# Autodesk Inventor assembly: wheeAndTrackLift
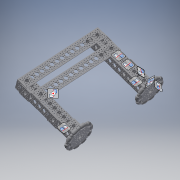
[picture p0: Inventor's stored thumbnail of the model, 180x180]
Saved by Autodesk Inventor 2017 (Build 210142000, 142)
## iProperties
Created: 2017-11-11
Part Number: wheeAndTrackLift
Document SubType Name: Assembly
Designer: User
Author: User
## Documents named in this file (5)
- C:\Robotics\CAD\2017-18_CAD\wheeAndTrackLift.iam
- C:\Robotics\CAD\COTSParts\Actobotics\585 parts\585450.ipt
- C:\Robotics\CAD\COTSParts\Actobotics\585 parts\585424.ipt
- C:\Robotics\CAD\COTSParts\Actobotics\595 parts\595671 Part.ipt
- C:\Robotics\CAD\COTSParts\Actobotics\585 parts\585728.ipt
## Components (12 placed, 4 different names)
1. 585450:1 — Flush:2, Mate:8, Mate:16, Flush:5, Mate:17, Flush:6, Mate:21, Mate:24, Mate:25, Mate:26, Flush:7, Mate:31, Mate:32
2. 585450:2 — Flush:2, Mate:10, Mate:16, Flush:4, Flush:5, Mate:18, Mate:19, Mate:20, Mate:22, Mate:23, Mate:27, Mate:28, Flush:8, Mate:29, Mate:30
3. 585424:1 — Mate:8, Mate:13, Mate:14, Mate:17, Flush:6
4. 585424:2 — Mate:10, Mate:11, Mate:12, Flush:4, Mate:18
5. 595671 Part:1 — Mate:13, Mate:14
6. 595671 Part:2 — Mate:11, Mate:12
7. 585728:1 — Mate:22, Mate:23, Mate:24
8. 585728:2 — Mate:19, Mate:20, Mate:21
9. 585424:3 — Mate:29, Mate:30, Flush:9, Flush:10
10. 585424:4 — Mate:31, Mate:32, Flush:10
11. 585424:5 — Mate:27, Mate:28, Flush:8, Flush:9
12. 585424:6 — Mate:25, Mate:26, Flush:7
## Relationships (31: Mate 23, Flush 8)
- Flush:2: 585450:1 ↔ 585450:2
- Mate:8: 585450:1 ↔ 585424:1
- Mate:10: 585450:2 ↔ 585424:2
- Mate:11: 585424:2 ↔ 595671 Part:2
- Mate:12: 585424:2 ↔ 595671 Part:2
- Mate:13: 585424:1 ↔ 595671 Part:1
- Mate:14: 585424:1 ↔ 595671 Part:1
- Mate:16 (228.6 mm): 585450:1 ↔ 585450:2
- Flush:4: 585450:2 ↔ 585424:2
- Flush:5: 585450:1 ↔ 585450:2
- Mate:17: 585450:1 ↔ 585424:1
- Flush:6: 585450:1 ↔ 585424:1
- Mate:18: 585450:2 ↔ 585424:2
- Mate:19: 585450:2 ↔ 585728:2
- Mate:20: 585450:2 ↔ 585728:2
- Mate:21: 585450:1 ↔ 585728:2
- Mate:22: 585450:2 ↔ 585728:1
- Mate:23: 585450:2 ↔ 585728:1
- Mate:24: 585450:1 ↔ 585728:1
- Mate:25: 585450:1 ↔ 585424:6
- Mate:26: 585450:1 ↔ 585424:6
- Flush:7: 585450:1 ↔ 585424:6
- Mate:27: 585450:2 ↔ 585424:5
- Mate:28: 585450:2 ↔ 585424:5
- Flush:8: 585450:2 ↔ 585424:5
- Mate:29: 585450:2 ↔ 585424:3
- Mate:30: 585450:2 ↔ 585424:3
- Flush:9: 585424:3 ↔ 585424:5
- Mate:31: 585450:1 ↔ 585424:4
- Mate:32: 585450:1 ↔ 585424:4
- Flush:10: 585424:3 ↔ 585424:4
